# Autodesk Inventor assembly: PCB enclosure_v2
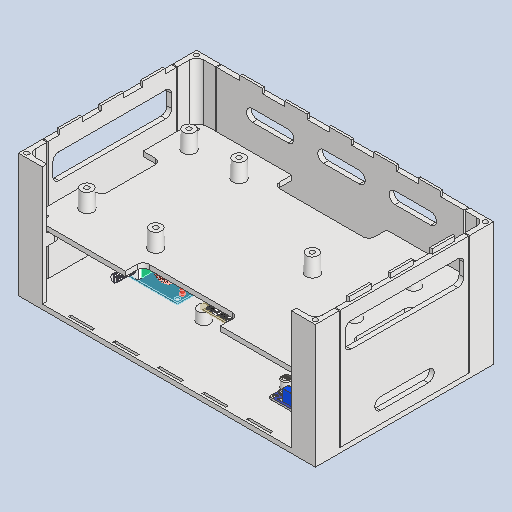
[picture p0: Inventor's stored thumbnail of the model, 512x512]
Saved by Autodesk Inventor 2026 (Build 300175050, 175E)
## iProperties
Created: 2025-10-28
Part Number: PCB enclosure_v2
Document SubType Name: Assembly
Designer: Kartik
Mass: 857.254 g
Surface Area: 6116.9 cm^2
Volume: 856.269 cm^3
Density: 1.00115 g/cm^3
Author: Kartik
## Documents named in this file (20)
- D:\Kartik\Projects\AMR\CAD\2 Sub-assembly\PCB enclosure_v2.iam
- D:\Kartik\Projects\AMR\CAD\4 Boughtouts\MDD20A CAD\MDD20A\MDD20A\MDD20A.ipt
- D:\Kartik\Projects\AMR\CAD\4 Boughtouts\NUCLEO-F401RE--3DModel-STEP-56544\NUCLEO-F401RE--3DModel-STEP-56544\NUCLEO-F401RE--3DModel-STEP-56544.ipt
- D:\Kartik\Projects\AMR\CAD\4 Boughtouts\nvidia-jetson-nano-4gb\Jetson nano 4GB\Jetson nano 4GB\Jetson nano 4GB.ipt
- D:\Kartik\Projects\AMR\CAD\4 Boughtouts\arduino-uno-screw-shield-1\Arduino Uno Screw Shield\Arduino Uno Screw Shield\Arduino Uno Screw Shield.ipt
- D:\Kartik\Projects\AMR\CAD\4 Boughtouts\xh-m401-buck-converter\XH-M401 Buck converter (XL4016E1)\XH-M401 Buck converter (XL4016E1)\XH-M401 Buck converter (XL4016E1).ipt
- D:\Kartik\Projects\AMR\CAD\4 Boughtouts\LM2596 DC-DC StepDown Converter v1\LM2596 DC-DC StepDown Converter v1\LM2596 DC-DC StepDown Converter v1.ipt
- D:\Kartik\Projects\AMR\CAD\4 Boughtouts\push-button-16-mm-led-1\LED_Button16mm\LED_Button_16mm\LED_Button_16mm\LED_Button_16mm.ipt
- D:\Kartik\Projects\AMR\CAD\4 Boughtouts\electrical-part-fuse-holder\Fuse Holder - CONQUER CQ-201N_.iam
- D:\Kartik\Projects\AMR\CAD\3 Parts\Enclosure_1.ipt
- D:\Kartik\Projects\AMR\CAD\4 Boughtouts\volt-meter-led-display-1\LED Display v3\LED Display v3\LED Display v3.ipt
- D:\Kartik\Projects\AMR\CAD\3 Parts\Enclosure_2.ipt
- D:\Kartik\Projects\AMR\CAD\3 Parts\Enclosure_4.ipt
- D:\Kartik\Projects\AMR\CAD\3 Parts\Enclosure_3.ipt
- D:\Kartik\Projects\AMR\CAD\3 Parts\Enclosure_5.ipt
- D:\Kartik\Projects\AMR\CAD\3 Parts\Enclosure_6.ipt
- D:\Kartik\Projects\AMR\CAD\3 Parts\Enclosure_7.ipt
- D:\Kartik\Projects\AMR\CAD\4 Boughtouts\volt-meter-led-display-1\LED Display v3\Amass XT60E1-M v4.ipt
- D:\Kartik\Projects\AMR\CAD\4 Boughtouts\mini-toggle-switches-1\6mm SPDT Mini Toggle Switch\6mm SPDT Mini Toggle Switch\6mm SPDT Mini Toggle Switch.ipt
- D:\Kartik\Projects\AMR\CAD\4 Boughtouts\emergency-stop-push-button-switches-ab6-v-series-16mm-1\AB6-V\AB6-V\AB6-V.ipt
## Components (19 placed, 19 different names)
1. MDD20A:1 — Flush:11, Mate:62, Mate:63, Angle:2
2. NUCLEO-F401RE--3DModel-STEP-56544:1 — Mate:25, Mate:26, Mate:27, Mate:67, Mate:68, Mate:69
3. Jetson nano 4GB:1 — Mate:64, Mate:65, Mate:66
4. Arduino Uno Screw Shield:1 — Mate:25, Mate:26, Mate:27
5. XH-M401 Buck converter (XL4016E1):1 — Flush:11
6. LM2596 DC-DC StepDown Converter v1:1 — Mate:70, Mate:71, Mate:72
7. LED_Button_16mm:1 — Flush:17, Mate:41, Flush:24
8. Fuse Holder - CONQUER CQ-201N_:2 [sub-assembly] — Mate:57, Mate:58, Angle:3
9. Enclosure_1:1 — Mate:32, Flush:18, Mate:33, Mate:34, Flush:19, Mate:35, Mate:36, Mate:37, Flush:20, Mate:38, Mate:39, Flush:21, Mate:40, Flush:23, Mate:46, Mate:62, Mate:63, Mate:70, Mate:71, Mate:72
10. LED Display v3:1 — Flush:17, Mate:42, Mate:43
11. Enclosure_2:1 — Mate:32, Flush:18, Mate:33, Flush:22, Angle:2
12. Enclosure_3:1 — Mate:34, Flush:19, Mate:35, Mate:44, Angle:3
13. Enclosure_4:1 — Mate:36, Mate:37, Flush:20
14. Enclosure_5:1 — Mate:38, Mate:39, Flush:21, Mate:45
15. Enclosure_6:1 — Mate:40, Flush:22, Flush:23, Mate:41, Flush:24, Mate:42, Mate:43, Mate:50, Mate:51, Mate:52, Mate:53, Mate:54, Mate:55, Mate:56, Mate:57, Mate:58
16. Enclosure_7:1 — Mate:44, Mate:45, Mate:46, Mate:64, Mate:65, Mate:66, Mate:67, Mate:68, Mate:69
17. Amass XT60E1-M v4:1 — Mate:54, Mate:55, Mate:56
18. 6mm SPDT Mini Toggle Switch:1 — Mate:50, Mate:51
19. AB6-V:1 — Mate:52, Mate:53
## Relationships (49: Mate 38, Flush 9, Angle 2)
- Mate:25: NUCLEO-F401RE--3DModel-STEP-56544:1 ↔ Arduino Uno Screw Shield:1
- Mate:26: NUCLEO-F401RE--3DModel-STEP-56544:1 ↔ Arduino Uno Screw Shield:1
- Mate:27: NUCLEO-F401RE--3DModel-STEP-56544:1 ↔ Arduino Uno Screw Shield:1
- Flush:11: MDD20A:1 ↔ XH-M401 Buck converter (XL4016E1):1
- Flush:17: LED_Button_16mm:1 ↔ LED Display v3:1
- Mate:32: Enclosure_1:1 ↔ Enclosure_2:1
- Flush:18: Enclosure_1:1 ↔ Enclosure_2:1
- Mate:33 (1 mm): Enclosure_1:1 ↔ Enclosure_2:1
- Mate:34: Enclosure_1:1 ↔ Enclosure_3:1
- Flush:19: Enclosure_1:1 ↔ Enclosure_3:1
- Mate:35 (1 mm): Enclosure_1:1 ↔ Enclosure_3:1
- Mate:36: Enclosure_1:1 ↔ Enclosure_4:1
- Mate:37 (1 mm): Enclosure_1:1 ↔ Enclosure_4:1
- Flush:20: Enclosure_1:1 ↔ Enclosure_4:1
- Mate:38: Enclosure_1:1 ↔ Enclosure_5:1
- Mate:39 (1 mm): Enclosure_1:1 ↔ Enclosure_5:1
- Flush:21: Enclosure_1:1 ↔ Enclosure_5:1
- Mate:40: Enclosure_1:1 ↔ Enclosure_6:1
- Flush:22: Enclosure_2:1 ↔ Enclosure_6:1
- Flush:23: Enclosure_1:1 ↔ Enclosure_6:1
- Mate:41: LED_Button_16mm:1 ↔ Enclosure_6:1
- Flush:24: LED_Button_16mm:1 ↔ Enclosure_6:1
- Mate:42: LED Display v3:1 ↔ Enclosure_6:1
- Mate:43: LED Display v3:1 ↔ Enclosure_6:1
- Mate:44 (1 mm): Enclosure_3:1 ↔ Enclosure_7:1
- Mate:45 (1 mm): Enclosure_5:1 ↔ Enclosure_7:1
- Mate:46: Enclosure_1:1 ↔ Enclosure_7:1
- Mate:50: Enclosure_6:1 ↔ 6mm SPDT Mini Toggle Switch:1
- Mate:51: Enclosure_6:1 ↔ 6mm SPDT Mini Toggle Switch:1
- Mate:52: Enclosure_6:1 ↔ AB6-V:1
- Mate:53: Enclosure_6:1 ↔ AB6-V:1
- Mate:54: Enclosure_6:1 ↔ Amass XT60E1-M v4:1
- Mate:55: Enclosure_6:1 ↔ Amass XT60E1-M v4:1
- Mate:56: Enclosure_6:1 ↔ Amass XT60E1-M v4:1
- Mate:57: Fuse Holder - CONQUER CQ-201N_:2 ↔ Enclosure_6:1
- Mate:58: Fuse Holder - CONQUER CQ-201N_:2 ↔ Enclosure_6:1
- Mate:62: MDD20A:1 ↔ Enclosure_1:1
- Mate:63 (1.5 mm): MDD20A:1 ↔ Enclosure_1:1
- Angle:2 (90 deg): MDD20A:1 ↔ Enclosure_2:1
- Mate:64: Jetson nano 4GB:1 ↔ Enclosure_7:1
- Mate:65: Jetson nano 4GB:1 ↔ Enclosure_7:1
- Mate:66: Jetson nano 4GB:1 ↔ Enclosure_7:1
- Angle:3 (0 deg): Fuse Holder - CONQUER CQ-201N_:2 ↔ Enclosure_3:1
- Mate:67: NUCLEO-F401RE--3DModel-STEP-56544:1 ↔ Enclosure_7:1
- Mate:68: NUCLEO-F401RE--3DModel-STEP-56544:1 ↔ Enclosure_7:1
- Mate:69: NUCLEO-F401RE--3DModel-STEP-56544:1 ↔ Enclosure_7:1
- Mate:70: LM2596 DC-DC StepDown Converter v1:1 ↔ Enclosure_1:1
- Mate:71: LM2596 DC-DC StepDown Converter v1:1 ↔ Enclosure_1:1
- Mate:72: LM2596 DC-DC StepDown Converter v1:1 ↔ Enclosure_1:1
